# Autodesk Inventor assembly: Assembly1
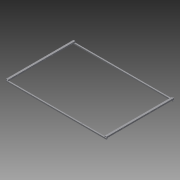
[picture p0: Inventor's stored thumbnail of the model, 180x180]
Saved by Autodesk Inventor 2015 SP1 (Build 190203100, 203)
## iProperties
Created: 2015-03-28
Part Number: Assembly1
Document SubType Name: Assembly
Designer: Cyril
Mass: 10678.5 g
Surface Area: 59183.2 cm^2
Volume: 10678.5 cm^3
Density: 1 g/cm^3
Author: Cyril
## Documents named in this file (5)
- C:\Users\Cyril\Documents\OSE FR\Concentrateur solaire\Inventor\Assemblage_Cadre.iam
- C:\Users\Cyril\Documents\OSE FR\Concentrateur solaire\Inventor\Part1.ipt
- C:\Users\Cyril\Documents\OSE FR\Concentrateur solaire\Inventor\Tube_50x40x2_L1430.ipt
- C:\Users\Cyril\Documents\OSE FR\Concentrateur solaire\Imported Components\test export STEP\test export STEP.ipt
- C:\Users\Cyril\Documents\OSE FR\Concentrateur solaire\Inventor\Bibliothèque\Imported Components\Hexagon_head_bolt_DINENISO4014_M6_65\Hexagon_head_bolt_DINENISO4014_M6_65.ipt
## Components (8 placed, 4 different names)
1. Part1:1 — Insert:1, Insert:2
2. Part1:2 — Insert:3, Insert:4, Insert:5, Insert:6, Flush:2, Insert:7, Insert:10
3. Tube_50x40x2_L1430:2 — Insert:5, Insert:6
4. Tube_50x40x2_L1430:1 — Insert:1, Insert:2, Insert:3, Insert:4, Flush:1, Flush:3, Insert:8, Insert:9
5. test export STEP:1 — Insert:7
6. test export STEP:2 — Insert:10
7. Hexagon_head_bolt_DINENISO4014_M6_65:1 — Insert:8
8. Hexagon_head_bolt_DINENISO4014_M6_65:2 — Insert:9
## Relationships (13: Insert 10, Flush 3)
- Insert:1: Part1:1 ↔ Tube_50x40x2_L1430:1
- Insert:2: Part1:1 ↔ Tube_50x40x2_L1430:1
- Insert:3: Part1:2 ↔ Tube_50x40x2_L1430:1
- Insert:4: Part1:2 ↔ Tube_50x40x2_L1430:1
- Insert:5: Part1:2 ↔ Tube_50x40x2_L1430:2
- Insert:6: Part1:2 ↔ Tube_50x40x2_L1430:2
- Flush:1: Tube_50x40x2_L1430:1
- Flush:2: Part1:2
- Flush:3: Tube_50x40x2_L1430:1
- Insert:7: Part1:2 ↔ test export STEP:1
- Insert:8: Tube_50x40x2_L1430:1 ↔ Hexagon_head_bolt_DINENISO4014_M6_65:1
- Insert:9: Tube_50x40x2_L1430:1 ↔ Hexagon_head_bolt_DINENISO4014_M6_65:2
- Insert:10: Part1:2 ↔ test export STEP:2
